# Autodesk Inventor assembly: Functioning swerve drive (CIM motor shaft)
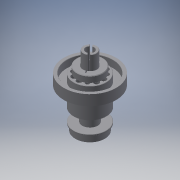
[picture p0: Inventor's stored thumbnail of the model, 180x180]
Saved by Autodesk Inventor 2019 (Build 230136000, 136)
## iProperties
Created: 2019-01-14
Part Number: Functioning swerve drive (CIM motor shaft)
Document SubType Name: Assembly
Designer: josh
Mass: 33.3455 g
Surface Area: 229.575 cm^2
Volume: 33.3455 cm^3
Density: 1 g/cm^3
Author: josh
## Documents named in this file (5)
- D:\Synthesis Robots\Epsilon\Functioning swerve drive sub-assemblies\Functioning swerve drive (CIM motor shaft).iam
- D:\Synthesis Robots\Epsilon\Swerve drive parts\FR8ZZ Bearing_smart.ipt
- D:\Synthesis Robots\Epsilon\Swerve drive parts\12T CIM Shaft.ipt
- D:\Synthesis Robots\Epsilon\Swerve drive parts\40T Sleeve Gear REV2.ipt
- D:\Synthesis Robots\Epsilon\Swerve drive parts\VEX 217-2736 0500 Collar Clamp.ipt
## Components (4 placed, 4 different names)
1. FR8ZZ Bearing_smart:2
2. 12T CIM Shaft:2 — Mate:16, Mate:18
3. 40T Sleeve Gear REV2:2 — Mate:17, Mate:18
4. VEX 217-2736 0500 Collar Clamp:2 — Mate:16, Mate:17
## Relationships (6: Mate 6)
- [Mate]: FR8ZZ Bearing_smart:2 ↔ 12T CIM Shaft:2
- [Mate]: FR8ZZ Bearing_smart:2 ↔ 12T CIM Shaft:2
- [Mate]: 12T CIM Shaft:2 ↔ 40T Sleeve Gear REV2:2
- Mate:16: 12T CIM Shaft:2 ↔ VEX 217-2736 0500 Collar Clamp:2
- Mate:17: 40T Sleeve Gear REV2:2 ↔ VEX 217-2736 0500 Collar Clamp:2
- Mate:18: 12T CIM Shaft:2 ↔ 40T Sleeve Gear REV2:2
## Named parameters: d23_d406_d216 = 0 mm, d24_d189_d93_d166 = 0 mm, d25_d309_d133_d165 = 0 mm
